# Autodesk Inventor assembly: bumper test
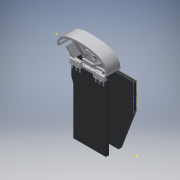
[picture p0: Inventor's stored thumbnail of the model, 180x180]
Saved by Autodesk Inventor 2016 (Build 200138000, 138)
## iProperties
Created: 2015-09-30
Part Number: bumper test
Document SubType Name: Assembly
Designer: Jesse Stevenson
Author: Jesse Stevenson
## Documents named in this file (7)
- C:\Users\Jesse Stevenson\Desktop\E-121-Design\bumper test.iam
- C:\Users\Jesse Stevenson\Desktop\E-121-Design\top.ipt
- C:\Users\Jesse Stevenson\Desktop\E-121-Design\bottom.ipt
- C:\Users\Jesse Stevenson\Desktop\E-121-Design\Microswitch_-_Omron_D2SW-P2L2T.iam
- C:\Users\Jesse Stevenson\Desktop\E-121-Design\bumper lever support.ipt
- C:\Users\Jesse Stevenson\Desktop\E-121-Design\lever2.ipt
- C:\Users\Jesse Stevenson\Desktop\E-121-Design\bumper.ipt
## Components (8 placed, 6 different names)
1. top:1 — Flush:1, Mate:1, Mate:2
2. bottom:1 — Flush:1, Mate:1, Mate:3, Flush:3, Flush:4, Mate:18, Mate:19, Angle:1
3. Microswitch_-_Omron_D2SW-P2L2T:1 [sub-assembly] — Flush:2, Mate:17, Mate:19
4. Microswitch_-_Omron_D2SW-P2L2T:2 [sub-assembly] — Flush:2, Mate:16, Mate:18, Angle:1
5. bumper lever support:1 — Flush:3, Flush:4, Mate:10, Mate:13, Mate:14
6. bumper:1 — Mate:8, Mate:9, Mate:11, Mate:15
7. lever2:1 — Mate:11, Mate:13, Mate:14, Mate:15, Mate:16
8. lever2:2 — Mate:8, Mate:9, Mate:10, Mate:17
## Relationships (20: Mate 15, Flush 4, Angle 1)
- Flush:1: top:1 ↔ bottom:1
- Mate:1 (18.923 mm): top:1 ↔ bottom:1
- Mate:2: top:1
- Mate:3: bottom:1
- Mate:4 (25.273 mm)
- Flush:2: Microswitch_-_Omron_D2SW-P2L2T:1 ↔ Microswitch_-_Omron_D2SW-P2L2T:2
- Flush:3: bottom:1 ↔ bumper lever support:1
- Flush:4: bottom:1 ↔ bumper lever support:1
- Mate:8: bumper:1 ↔ lever2:2
- Mate:9: bumper:1 ↔ lever2:2
- Mate:10: bumper lever support:1 ↔ lever2:2
- Mate:11: bumper:1 ↔ lever2:1
- Mate:13: bumper lever support:1 ↔ lever2:1
- Mate:14: bumper lever support:1 ↔ lever2:1
- Mate:15: bumper:1 ↔ lever2:1
- Mate:16 (-1.27 mm): Microswitch_-_Omron_D2SW-P2L2T:2 ↔ lever2:1
- Mate:17 (-1.27 mm): Microswitch_-_Omron_D2SW-P2L2T:1 ↔ lever2:2
- Mate:18: bottom:1 ↔ Microswitch_-_Omron_D2SW-P2L2T:2
- Mate:19: bottom:1 ↔ Microswitch_-_Omron_D2SW-P2L2T:1
- Angle:1 (0 deg): bottom:1 ↔ Microswitch_-_Omron_D2SW-P2L2T:2
